# Autodesk Inventor assembly: Robot B
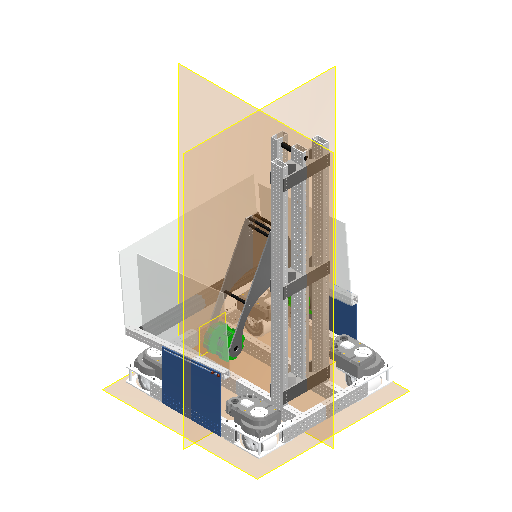
[picture p0: Inventor's stored thumbnail of the model, 512x512]
Saved by Autodesk Inventor 2025.3 (Build 293356000, 356)
## iProperties
Created: 2026-05-13
Part Number: Robot B
Document SubType Name: Assembly
Designer: djair.oliveira
Author: djair.oliveira
## Documents named in this file (5)
- C:\Users\djair.oliveira\Documents\GitHub\MT_2026\CAD\Model B\Robot B.iam
- C:\Users\djair.oliveira\Documents\GitHub\MT_2026\CAD\Model B\Chassi\Chassi.iam
- C:\Users\djair.oliveira\Documents\GitHub\MT_2026\CAD\Model B\Elevador\Elevador.iam
- C:\Users\djair.oliveira\Documents\GitHub\MT_2026\CAD\Model B\Hand\Hand.iam
- C:\Users\djair.oliveira\Documents\GitHub\MT_2026\CAD\Model B\Intake\Intake.iam
## Components (4 placed, 4 different names)
1. Chassi:1 [sub-assembly] — Coincidente:1, Alinhado:1, Alinhado:4, Coincidente:3, Coincidente:4, Coincidente:5, Tangente:1, Coincidente:7
2. Elevador:1 [sub-assembly] — Coincidente:1, Alinhado:1, Coincidente:2, Alinhado:3, Alinhado:4, Coincidente:6
3. Hand:1 [sub-assembly] — Coincidente:2, Alinhado:3
4. Intake:1 [sub-assembly] — Coincidente:3, Coincidente:4, Coincidente:5
## Relationships (11: Mate 7, Flush 3, Tangent 1)
- Coincidente:1 [Mate]: Chassi:1 ↔ Elevador:1
- Alinhado:1 [Flush]: Chassi:1 ↔ Elevador:1
- Coincidente:2 [Mate]: Elevador:1 ↔ Hand:1
- Alinhado:3 [Flush]: Elevador:1 ↔ Hand:1
- Alinhado:4 [Flush] (88.9 mm): Chassi:1 ↔ Elevador:1
- Coincidente:3 [Mate]: Chassi:1 ↔ Intake:1
- Coincidente:4 [Mate]: Chassi:1 ↔ Intake:1
- Coincidente:5 [Mate]: Chassi:1 ↔ Intake:1
- Tangente:1: Chassi:1
- Coincidente:6 [Mate] (76.2 mm): Elevador:1
- Coincidente:7 [Mate] (-292.1 mm): Chassi:1
